# Autodesk Inventor assembly: Assembly2
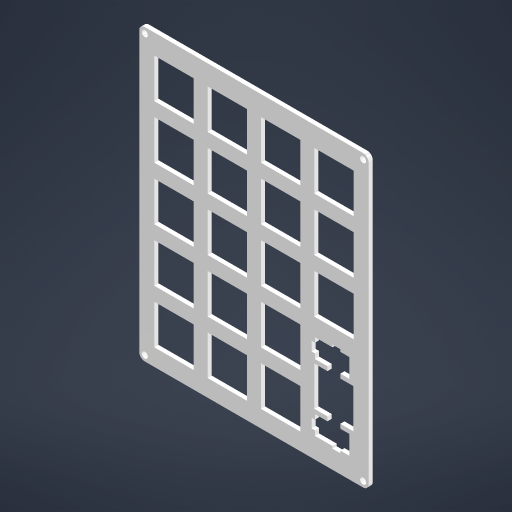
[picture p0: Inventor's stored thumbnail of the model, 512x512]
Saved by Autodesk Inventor 2024.2 (Build 282272000, 272)
## iProperties
Created: 2025-05-21
Part Number: Assembly2
Document SubType Name: Assembly
Designer: Moe
Author: Moe
## Documents named in this file (2)
- D:\Code\git\Model-C\case\Assembly2.iam
- D:\Code\git\Model-C\case\switchplate.ipt
## Components (1 placed, 1 different names)
1. switchplate:1
## Named parameters: Finish1_Area = 113.144
note: some values were not read from the file. Shown as the stored number, unit unknown: "Finish1_Area".
